# Autodesk Inventor assembly: square_one
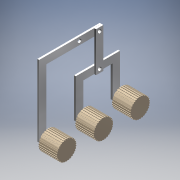
[picture p0: Inventor's stored thumbnail of the model, 180x180]
Saved by Autodesk Inventor 2018.1 (Build 221171000, 171)
## iProperties
Created: 2017-10-26
Part Number: square_one
Material: 一般
Document SubType Name: Assembly
Designer: Kakeru Yamashita
Author: Kakeru Yamashita
## Documents named in this file (5)
- C:\Users\Kakeru Yamashita\Documents\Inventor\Rocker_bogie_sim\square_one.iam
- C:\Users\Kakeru Yamashita\Documents\Inventor\Rocker_bogie_sim\tire.ipt
- C:\Users\Kakeru Yamashita\Documents\Inventor\Rocker_bogie_sim\bogie_square.ipt
- C:\Users\Kakeru Yamashita\Documents\Inventor\Rocker_bogie_sim\rocker.ipt
- C:\Users\Kakeru Yamashita\Documents\Inventor\Rocker_bogie_sim\rocker_bogie_plate.ipt
## Components (6 placed, 4 different names)
1. tire:1 — フラッシュ:1, メイト:2, フラッシュ:2
2. tire:2 — フラッシュ:1, メイト:1, フラッシュ:5
3. bogie_square:1 — メイト:1, メイト:2, フラッシュ:2, メイト:4, メイト:7
4. rocker:1 — メイト:3, フラッシュ:6, メイト:5, メイト:6, フラッシュ:7
5. tire:3 — フラッシュ:5, メイト:3, フラッシュ:6
6. rocker_bogie_plate:1 — メイト:4, メイト:5, メイト:6, メイト:7, フラッシュ:7
## Relationships (12: Mate 7, Flush 5)
- フラッシュ:1 [Flush]: tire:1 ↔ tire:2
- メイト:1 [Mate]: tire:2 ↔ bogie_square:1
- メイト:2 [Mate]: tire:1 ↔ bogie_square:1
- フラッシュ:2 [Flush]: tire:1 ↔ bogie_square:1
- フラッシュ:5 [Flush]: tire:2 ↔ tire:3
- メイト:3 [Mate]: rocker:1 ↔ tire:3
- フラッシュ:6 [Flush]: rocker:1 ↔ tire:3
- メイト:4 [Mate]: bogie_square:1 ↔ rocker_bogie_plate:1
- メイト:5 [Mate]: rocker:1 ↔ rocker_bogie_plate:1
- メイト:6 [Mate]: rocker:1 ↔ rocker_bogie_plate:1
- メイト:7 [Mate]: bogie_square:1 ↔ rocker_bogie_plate:1
- フラッシュ:7 [Flush]: rocker:1 ↔ rocker_bogie_plate:1
